# Autodesk Inventor assembly: Assembly
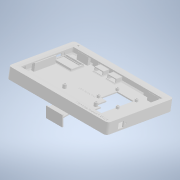
[picture p0: Inventor's stored thumbnail of the model, 180x180]
Saved by Autodesk Inventor 2021 (Build 250183000, 183)
## iProperties
Created: 2020-06-15
Part Number: Assembly
Document SubType Name: Assembly
Designer: Mariano
Author: Mariano
## Documents named in this file (4)
- D:\Source\SvnDocuments\Projects\ELinkDisplay\Assembly.iam
- D:\Source\SvnDocuments\Projects\ELinkDisplay\Bottom.ipt
- D:\Source\SvnDocuments\Projects\ELinkDisplay\Top.ipt
- D:\Source\SvnDocuments\Projects\ELinkDisplay\Holder.ipt
## Components (3 placed, 3 different names)
1. Bottom:1 — Flush:1, Flush:2, Mate:1, Mate:2, Mate:3, Flush:3
2. Top:1 — Flush:1, Flush:2, Mate:1
3. Holder:1 — Mate:2, Mate:3, Flush:3
## Relationships (6: Flush 3, Mate 3)
- Flush:1: Bottom:1 ↔ Top:1
- Flush:2: Bottom:1 ↔ Top:1
- Mate:1: Bottom:1 ↔ Top:1
- Mate:2: Bottom:1 ↔ Holder:1
- Mate:3: Bottom:1 ↔ Holder:1
- Flush:3: Bottom:1 ↔ Holder:1
